# Autodesk Inventor assembly: DN35CF 4SMA
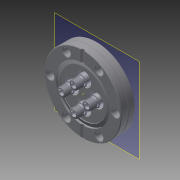
[picture p0: Inventor's stored thumbnail of the model, 180x180]
Saved by Autodesk Inventor 2015 (Build 190159000, 159)
## iProperties
Created: 2014-05-19
Part Number: DN35CF 4SMA
Document SubType Name: Assembly
Designer: jad211
Author: jad211
## Documents named in this file (3)
- C:\CADFiles\Generic vacuum components\DN35CF 4SMA.iam
- C:\CADFiles\Generic vacuum components\DN35CF Blank.ipt
- C:\CADFiles\Generic vacuum components\Imported Components\ifdcg012013\F0275X0501P_3.ipt
## Components (5 placed, 2 different names)
1. DN35CF Blank:1 — Flush:1, Mate:1, Insert:1, Insert:2, Insert:3, Insert:4
2. F0275X0501P_3:1 — Insert:1
3. F0275X0501P_3:2 — Insert:2
4. F0275X0501P_3:3 — Insert:4
5. F0275X0501P_3:4 — Insert:3
## Relationships (6: Insert 4, Flush 1, Mate 1)
- Flush:1: DN35CF Blank:1
- Mate:1: DN35CF Blank:1
- Insert:1: DN35CF Blank:1 ↔ F0275X0501P_3:1
- Insert:2: DN35CF Blank:1 ↔ F0275X0501P_3:2
- Insert:3: DN35CF Blank:1 ↔ F0275X0501P_3:4
- Insert:4: DN35CF Blank:1 ↔ F0275X0501P_3:3
